# Autodesk Inventor assembly: ankle_w_feet_left
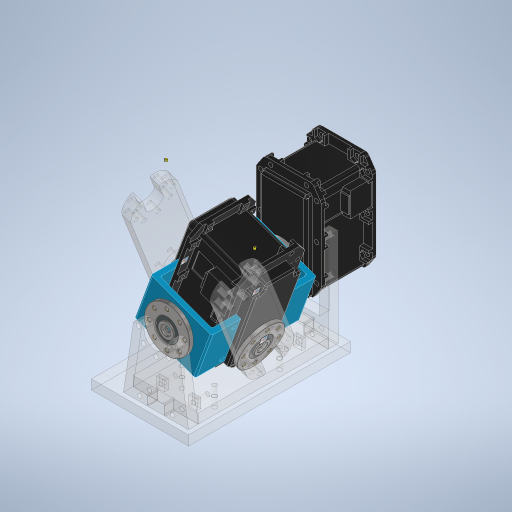
[picture p0: Inventor's stored thumbnail of the model, 512x512]
Saved by Autodesk Inventor 2024 (Build 280153000, 153)
## iProperties
Created: 2024-09-16
Part Number: ankle_w_feet_left
Document SubType Name: Assembly
Designer: jmha0
Author: jmha0
## Documents named in this file (13)
- C:\Users\jmha0\OneDrive\바탕 화면\19th_intern_hjm_fight_robot\부품\Lower_Body\ankle_w_feet\ankle_w_feet_right.iam
- C:\Users\jmha0\OneDrive\바탕 화면\19th_intern_hjm_fight_robot\부품\Lower_Body\feet\feet.ipt
- C:\Users\jmha0\OneDrive\바탕 화면\19th_intern_hjm_fight_robot\부품\Lower_Body\feet\feet_holder1.ipt
- C:\Users\jmha0\OneDrive\바탕 화면\19th_intern_hjm_fight_robot\부품\Lower_Body\feet\feet_holder2.ipt
- C:\Users\jmha0\OneDrive\바탕 화면\19th_intern_hjm_fight_robot\부품\Lower_Body\feet\feet_holder3.ipt
- C:\Users\jmha0\OneDrive\바탕 화면\19th_intern_hjm_fight_robot\부품\hardware\ROBOTIS(Inventor 2024 ver.)\아이들러\64아이들러.iam
- C:\Users\jmha0\OneDrive\바탕 화면\19th_intern_hjm_fight_robot\부품\Lower_Body\ankle_w_motor\3D_ankle1.ipt
- C:\Users\jmha0\OneDrive\바탕 화면\19th_intern_hjm_fight_robot\부품\Lower_Body\ankle_w_motor\3D_ankle2.ipt
- C:\Users\jmha0\OneDrive\바탕 화면\19th_intern_hjm_fight_robot\부품\hardware\ROBOTIS(Inventor 2024 ver.)\다이나믹셀\MX-64T.ipt
- C:\Users\jmha0\OneDrive\바탕 화면\19th_intern_hjm_fight_robot\부품\hardware\ROBOTIS(Inventor 2024 ver.)\혼\64-106Horn.ipt
- C:\Users\jmha0\OneDrive\바탕 화면\19th_intern_hjm_fight_robot\부품\hardware\ROBOTIS(Inventor 2024 ver.)\다이나믹셀\MX-106T+idle.ipt.iam
- C:\Users\jmha0\OneDrive\바탕 화면\19th_intern_hjm_fight_robot\부품\Lower_Body\knee_w_motor\frame_ankle_to_knee1.ipt
- MX-106T+idle.ipt
## Components (13 placed, 11 different names)
1. feet:1 — 삽입:1, 삽입:2, 삽입:3, 삽입:4
2. feet_holder1:1 — 삽입:5, 삽입:6, 메이트:1, 각도:1
3. feet_holder2:1 — 삽입:7, 삽입:8, 삽입:10, 삽입:11, 삽입:12, 삽입:13
4. feet_holder3:1 — 삽입:1, 삽입:2, 삽입:3, 삽입:4, 삽입:5, 삽입:6, 삽입:7, 삽입:8, 각도:9
5. 64아이들러:1 [sub-assembly] — 메이트:1, 각도:1, 메이트:2, 각도:2
6. 3D_ankle1:1 — 메이트:2, 각도:2, 삽입:25, 삽입:27
7. 3D_ankle2:1 — 삽입:22, 삽입:24, 삽입:26
8. MX-64T:1 — 삽입:10, 삽입:11, 삽입:12, 삽입:13
9. 64-106Horn:1 — 삽입:22
10. frame_ankle_to_knee1:1 — 메이트:3, 각도:5, 각도:6, 각도:7, 각도:8
11. frame_ankle_to_knee1:2 — 메이트:4, 각도:6, 각도:7
12. 64-106Horn:2 — 삽입:23, 메이트:4
13. MX-106T+idle.ipt:1 [sub-assembly] — 삽입:23, 삽입:24, 삽입:25, 삽입:26, 삽입:27, 메이트:3, 각도:5, 각도:8, 각도:9
## Relationships (29: Insert 18, Angle 7, Mate 4)
- 삽입:1 [Insert]: feet:1 ↔ feet_holder3:1
- 삽입:2 [Insert]: feet:1 ↔ feet_holder3:1
- 삽입:3 [Insert]: feet:1 ↔ feet_holder3:1
- 삽입:4 [Insert]: feet:1 ↔ feet_holder3:1
- 삽입:5 [Insert]: feet_holder1:1 ↔ feet_holder3:1
- 삽입:6 [Insert]: feet_holder1:1 ↔ feet_holder3:1
- 삽입:7 [Insert]: feet_holder2:1 ↔ feet_holder3:1
- 삽입:8 [Insert]: feet_holder2:1 ↔ feet_holder3:1
- 메이트:1 [Mate]: feet_holder1:1 ↔ 64아이들러:1
- 각도:1 [Angle] (0 deg): feet_holder1:1 ↔ 64아이들러:1
- 삽입:10 [Insert] (2 mm): feet_holder2:1 ↔ MX-64T:1
- 삽입:11 [Insert] (2 mm): feet_holder2:1 ↔ MX-64T:1
- 삽입:12 [Insert] (2 mm): feet_holder2:1 ↔ MX-64T:1
- 삽입:13 [Insert] (2 mm): feet_holder2:1 ↔ MX-64T:1
- 메이트:2 [Mate]: 64아이들러:1 ↔ 3D_ankle1:1
- 삽입:22 [Insert]: 3D_ankle2:1 ↔ 64-106Horn:1
- 각도:2 [Angle] (0 deg): 64아이들러:1 ↔ 3D_ankle1:1
- 삽입:23 [Insert] (0.1 mm): 64-106Horn:2 ↔ MX-106T+idle.ipt:1
- 삽입:24 [Insert]: 3D_ankle2:1 ↔ MX-106T+idle.ipt:1
- 삽입:25 [Insert]: 3D_ankle1:1 ↔ MX-106T+idle.ipt:1
- 삽입:26 [Insert]: 3D_ankle2:1 ↔ MX-106T+idle.ipt:1
- 삽입:27 [Insert]: 3D_ankle1:1 ↔ MX-106T+idle.ipt:1
- 메이트:3 [Mate]: frame_ankle_to_knee1:1 ↔ MX-106T+idle.ipt:1
- 메이트:4 [Mate]: frame_ankle_to_knee1:2 ↔ 64-106Horn:2
- 각도:5 [Angle] (0 deg): frame_ankle_to_knee1:1 ↔ MX-106T+idle.ipt:1
- 각도:6 [Angle] (0 deg): frame_ankle_to_knee1:1 ↔ frame_ankle_to_knee1:2
- 각도:7 [Angle] (0 deg): frame_ankle_to_knee1:1 ↔ frame_ankle_to_knee1:2
- 각도:8 [Angle] (30 deg): frame_ankle_to_knee1:1 ↔ MX-106T+idle.ipt:1
- 각도:9 [Angle] (200 deg): feet_holder3:1 ↔ MX-106T+idle.ipt:1
